# Autodesk Inventor assembly: gasienica_zlozenie
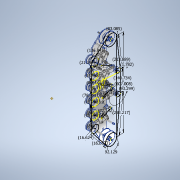
[picture p0: Inventor's stored thumbnail of the model, 180x180]
Saved by Autodesk Inventor 2020.3 (Build 243373000, 373)
## iProperties
Created: 2021-10-24
Part Number: gasienica_zlozenie
Document SubType Name: Assembly
Designer: patry
Author: patry
## Documents named in this file (31)
- C:\Users\patry\Desktop\Konar staff\Ariadna2.1\ariadna_mechanika\Obszar roboczy\Naped\Zawieszenie_v3\gasienica_zlozenie.iam
- C:\Users\patry\Desktop\Konar staff\Ariadna2.1\ariadna_mechanika\Obszar roboczy\Naped\Zawieszenie_v3\plyta_glowna_V3.ipt
- C:\Users\patry\Desktop\Konar staff\Ariadna2.1\ariadna_mechanika\Obszar roboczy\Naped\Sruby\M6_nut_5mm_MIR1.ipt
- C:\Users\patry\Desktop\Konar staff\Ariadna2.1\ariadna_mechanika\Obszar roboczy\Naped\Sruby\M6x65_MIR1.ipt
- C:\Users\patry\Desktop\Konar staff\Ariadna2.1\ariadna_mechanika\Obszar roboczy\Naped\Kola\kolo_przednie.iam
- C:\Users\patry\Desktop\Konar staff\Ariadna2.1\ariadna_mechanika\Obszar roboczy\Naped\Sruby\M5x65.ipt
- C:\Users\patry\Desktop\Konar staff\Ariadna2.1\ariadna_mechanika\Obszar roboczy\Naped\Sruby\M5_nut_5mm.ipt
- C:\Users\patry\Desktop\Konar staff\Ariadna2.1\ariadna_mechanika\Obszar roboczy\Naped\Sruby\dystans_miedzy_plytami.ipt
- C:\Users\patry\Desktop\Konar staff\Ariadna2.1\ariadna_mechanika\Obszar roboczy\Naped\Zawieszenie_v3\glowny_wahacz.ipt
- C:\Users\patry\Desktop\Konar staff\Ariadna2.1\ariadna_mechanika\Obszar roboczy\Naped\Zawieszenie_v3\ramie_1_wahacza.ipt
- C:\Users\patry\Desktop\Konar staff\Ariadna2.1\ariadna_mechanika\Obszar roboczy\Naped\Zawieszenie_v3\ramie_2_wahacza.ipt
- C:\Users\patry\Desktop\Konar staff\Ariadna2.1\ariadna_mechanika\Obszar roboczy\Naped\Zawieszenie_v3\tuleja_TUF106040.ipt
- C:\Users\patry\Desktop\Konar staff\Ariadna2.1\ariadna_mechanika\Obszar roboczy\Naped\Zawieszenie_v3\komplet_kol_V4.iam
- C:\Users\patry\Desktop\Konar staff\Ariadna2.1\ariadna_mechanika\Obszar roboczy\Naped\Sruby\M6_nut_5mm.ipt
- C:\Users\patry\Desktop\Konar staff\Ariadna2.1\ariadna_mechanika\Obszar roboczy\Naped\Sruby\M6x20.ipt
- C:\Users\patry\Desktop\Konar staff\Ariadna2.1\ariadna_mechanika\Obszar roboczy\Naped\Sruby\M6x65.ipt
- C:\Users\patry\Desktop\Konar staff\Ariadna2.1\ariadna_mechanika\Obszar roboczy\Naped\Zawieszenie_v3\independent_wheel_pair.iam
- C:\Users\patry\Desktop\Konar staff\Ariadna2.1\ariadna_mechanika\Obszar roboczy\Naped\Sruby\M6x35.ipt
- C:\Users\patry\Desktop\Konar staff\Ariadna2.1\ariadna_mechanika\Obszar roboczy\Naped\Amortyzator\Korpus.ipt
- C:\Users\patry\Desktop\Konar staff\Ariadna2.1\ariadna_mechanika\Obszar roboczy\Naped\Amortyzator\Tlok.ipt
- C:\Users\patry\Desktop\Konar staff\Ariadna2.1\ariadna_mechanika\Obszar roboczy\Naped\Amortyzator\Nakretka.ipt
- C:\Users\patry\Desktop\Konar staff\Ariadna2.1\ariadna_mechanika\Obszar roboczy\Naped\Sruby\M3_nut_5mm.ipt
- C:\Users\patry\Desktop\Konar staff\Ariadna2.1\ariadna_mechanika\Obszar roboczy\Naped\Sruby\M3x30.ipt
- C:\Users\patry\Desktop\Konar staff\Ariadna2.1\ariadna_mechanika\Obszar roboczy\Naped\Kola\single_wheel_dummie.iam
- C:\Users\patry\Desktop\Konar staff\Ariadna2.1\ariadna_mechanika\Obszar roboczy\Naped\Sruby\M5x40_threaded.ipt
- C:\Users\patry\Desktop\Konar staff\Ariadna2.1\ariadna_mechanika\Obszar roboczy\Naped\Zawieszenie_v3\glowny_wahacz_zewn.ipt
- C:\Users\patry\Desktop\Konar staff\Ariadna2.1\ariadna_mechanika\Obszar roboczy\Naped\Sruby\M8_nut_6.5mm_MIR1.ipt
- C:\Users\patry\Desktop\Konar staff\Ariadna2.1\ariadna_mechanika\Obszar roboczy\Naped\Sruby\M8x80_threaded_MIR1.ipt
- C:\Users\patry\Desktop\Konar staff\Ariadna2.1\ariadna_mechanika\Obszar roboczy\Naped\Sruby\M8_pad_MIR1.ipt
- C:\Users\patry\Desktop\Konar staff\Ariadna2.1\ariadna_mechanika\Obszar roboczy\Naped\Lozyska\608ZZ-8mm\bearings-608zz-80018-1.snapshot.1\608zz_MIR1.ipt
- C:\Users\patry\Desktop\Konar staff\Ariadna2.1\ariadna_mechanika\Obszar roboczy\Naped\Kola\kolo_napedowe.iam
## Components (177 placed, 30 different names)
1. plyta_glowna_V3:1 — Zestawiające:1, Zestawiające:2, Zestawiające:3, Zestawiające:107, Zestawiające:108, Zestawiające:110, Zestawiające:190, Zestawiające:191, Kątowe:20, Zestawiające:193, Zestawiające:260, Zestawiające:261, Zestawiające:263, Zestawiające:330, Zestawiające:331, Zestawiające:332, Zestawiające:333
2. plyta_glowna_V3:2 — Zestawiające:1, Zestawiające:2, Zestawiające:3, Zestawiające:11, Zestawiające:12, Zestawiające:19, Zestawiające:20, Zestawiające:21, Zestawiające:22, Zestawiające:26, Zestawiające:27, Zestawiające:109, Zestawiające:192, Zestawiające:262, Zestawiające:354, Równoległe:15, Kątowe:43
3. M6_nut_5mm_MIR1:1
4. M6x65_MIR1:1 — Zestawiające:11, Zestawiające:12
5. M6_nut_5mm_MIR1:2
6. M6_nut_5mm_MIR1:3
7. kolo_przednie:1 [sub-assembly]
8. M5x65:1 — Zestawiające:14, Zestawiające:15, Zestawiające:19, Zestawiające:20
9. M5_nut_5mm:1
10. dystans_miedzy_plytami:1 — Zestawiające:14, Zestawiające:15
11. M5x65:2 — Zestawiające:21, Zestawiające:22
12. M5_nut_5mm:2
13. dystans_miedzy_plytami:2
14. M5x65:3 — Zestawiające:26, Zestawiające:27
15. M5_nut_5mm:3
16. dystans_miedzy_plytami:3
17. glowny_wahacz:1
18. ramie_1_wahacza:1
19. ramie_2_wahacza:1
20. tuleja_TUF106040:1
21. tuleja_TUF106040:2
22. tuleja_TUF106040:3
23. tuleja_TUF106040:4
24. komplet_kol_V4:1 [sub-assembly] — Kątowe:43
25. glowny_wahacz:2 — Kątowe:40
26. ramie_1_wahacza:2 — Kątowe:40
27. tuleja_TUF106040:5
28. tuleja_TUF106040:6
29. ramie_2_wahacza:2
30. tuleja_TUF106040:7
31. tuleja_TUF106040:8
32. M6_nut_5mm:1
33. M6x20:1
34. M6_nut_5mm:2
35. M6_nut_5mm:3
36. M6_nut_5mm:4
37. M6x65:1 — Zestawiające:107
38. M6_nut_5mm:5
39. M6_nut_5mm:6
40. M6_nut_5mm:7
41. M6x65:2 — Zestawiające:108, Zestawiające:109
42. M6_nut_5mm:8
43. M6_nut_5mm:9
44. M6x35:1
45. M6x35:2
46. Korpus:1 — Walcowe:1
47. Tlok:1 — Walcowe:1
48. Nakretka:1
49. M3_nut_5mm:1
50. M3x30:1
51. M5_nut_5mm:4
52. M5x65:4 — Zestawiające:110
53. single_wheel_dummie:1 [sub-assembly]
54. M5_nut_5mm:5
55. M5x40_threaded:1
56. single_wheel_dummie:2 [sub-assembly]
57. M5_nut_5mm:6
58. glowny_wahacz:3
59. ramie_1_wahacza:3
60. ramie_2_wahacza:3
61. tuleja_TUF106040:9
62. tuleja_TUF106040:10
63. tuleja_TUF106040:11
64. tuleja_TUF106040:12
65. komplet_kol_V4:2 [sub-assembly] — Kątowe:20
66. glowny_wahacz:4 — Kątowe:41
67. ramie_1_wahacza:4 — Kątowe:41
68. tuleja_TUF106040:13
69. tuleja_TUF106040:14
70. ramie_2_wahacza:4
71. tuleja_TUF106040:15
72. tuleja_TUF106040:16
73. M6_nut_5mm:10
74. M6x20:2
75. M6_nut_5mm:11
76. M6_nut_5mm:12
77. M6_nut_5mm:13
78. M6x65:3 — Zestawiające:191, Zestawiające:192
79. M6_nut_5mm:14
80. M6_nut_5mm:15
81. M6_nut_5mm:16
82. M6x65:4 — Zestawiające:190
83. M6_nut_5mm:17
84. M6_nut_5mm:18
85. M6x35:3
86. M6x35:4
87. Korpus:2 — Walcowe:2
88. Tlok:2 — Walcowe:2
89. Nakretka:2
90. M3_nut_5mm:2
91. M3x30:2
92. M5_nut_5mm:7
93. M5x65:5 — Zestawiające:193
94. single_wheel_dummie:3 [sub-assembly]
95. M5_nut_5mm:8
96. M5x40_threaded:2
97. single_wheel_dummie:4 [sub-assembly]
98. M5_nut_5mm:9
99. ramie_1_wahacza:5 — Kątowe:39
100. ramie_2_wahacza:5
101. tuleja_TUF106040:17
102. tuleja_TUF106040:18
103. tuleja_TUF106040:19
104. tuleja_TUF106040:20
105. ramie_1_wahacza:6
106. tuleja_TUF106040:21
107. tuleja_TUF106040:22
108. ramie_2_wahacza:6
109. tuleja_TUF106040:23
110. tuleja_TUF106040:24
111. M6_nut_5mm:19
112. M6_nut_5mm:20
113. M6_nut_5mm:21
114. M6x65:5 — Zestawiające:260
115. M6_nut_5mm:22
116. M6_nut_5mm:23
117. M6_nut_5mm:24
118. M6x65:6 — Zestawiające:261
119. M6_nut_5mm:25 — Zestawiające:262
120. M6_nut_5mm:26
121. M6x35:5
122. M6x35:6
123. Korpus:3 — Walcowe:3
124. Tlok:3 — Walcowe:3
125. Nakretka:3
126. M3_nut_5mm:3
127. M3x30:3
128. M5_nut_5mm:10
129. M5x65:6 — Zestawiające:263
130. glowny_wahacz_zewn:1
131. glowny_wahacz_zewn:2 — Kątowe:39
132. independent_wheel_pair:1 [sub-assembly]
133. ramie_1_wahacza:7 — Kątowe:42
134. ramie_2_wahacza:7
135. tuleja_TUF106040:25
136. tuleja_TUF106040:26
137. tuleja_TUF106040:27
138. tuleja_TUF106040:28
139. ramie_1_wahacza:8
140. tuleja_TUF106040:29
141. tuleja_TUF106040:30
142. ramie_2_wahacza:8
143. tuleja_TUF106040:31
144. tuleja_TUF106040:32
145. M6_nut_5mm:27
146. M6_nut_5mm:28
147. M6_nut_5mm:29
148. M6x65:7 — Zestawiające:330
149. M6_nut_5mm:30 — Zestawiające:331
150. M6_nut_5mm:31
151. M6_nut_5mm:32
152. M6x65:8 — Zestawiające:332
153. M6_nut_5mm:33
154. M6_nut_5mm:34
155. M6x35:7
156. M6x35:8
157. Korpus:4 — Walcowe:4
158. Tlok:4 — Walcowe:4
159. Nakretka:4
160. M3_nut_5mm:4
161. M3x30:4
162. M5_nut_5mm:11
163. M5x65:7 — Zestawiające:333
164. glowny_wahacz_zewn:3
165. glowny_wahacz_zewn:4 — Kątowe:42
166. independent_wheel_pair:2 [sub-assembly]
167. M8_nut_6.5mm_MIR1:1
168. M8x80_threaded_MIR1:1
169. M8_nut_6.5mm_MIR1:2
170. M8_nut_6.5mm_MIR1:3
171. M8_pad_MIR1:1
172. M8_pad_MIR1:2
173. M8_pad_MIR1:3
174. M8_pad_MIR1:4
175. 608zz_MIR1:1
176. 608zz_MIR1:2 — Zestawiające:354, Równoległe:15
177. kolo_napedowe:1 [sub-assembly]
## Relationships (415: Mate 354, Angle 42, Flush 15, CylindricalJoint 4)
- Zestawiające:1 [Mate]: plyta_glowna_V3:1 ↔ plyta_glowna_V3:2
- Zestawiające:2 [Mate]: plyta_glowna_V3:1 ↔ plyta_glowna_V3:2
- Zestawiające:3 [Mate] (50 mm): plyta_glowna_V3:1 ↔ plyta_glowna_V3:2
- [Flush]: M6_nut_5mm_MIR1:1 ↔ M6x65_MIR1:1
- [Mate]: M6_nut_5mm_MIR1:1 ↔ M6x65_MIR1:1
- [Mate] (12 mm): M6_nut_5mm_MIR1:1 ↔ M6_nut_5mm_MIR1:2
- [Mate]: M6x65_MIR1:1 ↔ M6_nut_5mm_MIR1:2
- [Mate] (12 mm): M6x65_MIR1:1 ↔ M6_nut_5mm_MIR1:3
- [Mate]: M6x65_MIR1:1 ↔ M6_nut_5mm_MIR1:3
- [Mate]: M6x65_MIR1:1 ↔ kolo_przednie:1
- [Mate]: M6_nut_5mm_MIR1:3 ↔ kolo_przednie:1
- Zestawiające:11 [Mate]: plyta_glowna_V3:2 ↔ M6x65_MIR1:1
- Zestawiające:12 [Mate]: plyta_glowna_V3:2 ↔ M6x65_MIR1:1
- [Mate]: M5x65:1 ↔ M5_nut_5mm:1
- [Flush]: M5x65:1 ↔ M5_nut_5mm:1
- Zestawiające:14 [Mate]: M5x65:1 ↔ dystans_miedzy_plytami:1
- Zestawiające:15 [Mate] (5 mm): M5x65:1 ↔ dystans_miedzy_plytami:1
- [Mate]: M5x65:2 ↔ M5_nut_5mm:2
- [Flush]: M5x65:2 ↔ M5_nut_5mm:2
- [Mate]: M5x65:2 ↔ dystans_miedzy_plytami:2
- [Mate] (5 mm): M5x65:2 ↔ dystans_miedzy_plytami:2
- Zestawiające:19 [Mate]: plyta_glowna_V3:2 ↔ M5x65:1
- Zestawiające:20 [Mate]: plyta_glowna_V3:2 ↔ M5x65:1
- Zestawiające:21 [Mate]: plyta_glowna_V3:2 ↔ M5x65:2
- Zestawiające:22 [Mate]: plyta_glowna_V3:2 ↔ M5x65:2
- [Mate]: M5x65:3 ↔ M5_nut_5mm:3
- [Flush]: M5x65:3 ↔ M5_nut_5mm:3
- [Mate]: M5x65:3 ↔ dystans_miedzy_plytami:3
- [Mate] (5 mm): M5x65:3 ↔ dystans_miedzy_plytami:3
- Zestawiające:26 [Mate]: plyta_glowna_V3:2 ↔ M5x65:3
- Zestawiające:27 [Mate]: plyta_glowna_V3:2 ↔ M5x65:3
- [Mate]: ramie_2_wahacza:1 ↔ tuleja_TUF106040:1
- [Mate]: ramie_2_wahacza:1 ↔ tuleja_TUF106040:1
- [Mate]: ramie_2_wahacza:1 ↔ tuleja_TUF106040:2
- [Mate]: ramie_2_wahacza:1 ↔ tuleja_TUF106040:2
- [Angle] (0 deg): ramie_2_wahacza:1 ↔ tuleja_TUF106040:1
- [Angle] (0 deg): ramie_2_wahacza:1 ↔ tuleja_TUF106040:2
- [Mate]: ramie_1_wahacza:1 ↔ tuleja_TUF106040:3
- [Mate]: ramie_1_wahacza:1 ↔ tuleja_TUF106040:3
- [Angle] (0 deg): ramie_1_wahacza:1 ↔ tuleja_TUF106040:3
- [Mate]: ramie_1_wahacza:1 ↔ tuleja_TUF106040:4
- [Mate]: ramie_1_wahacza:1 ↔ tuleja_TUF106040:4
- [Angle] (0 deg): ramie_1_wahacza:1 ↔ tuleja_TUF106040:4
- [Mate]: glowny_wahacz:1 ↔ komplet_kol_V4:1
- [Mate]: komplet_kol_V4:1 ↔ glowny_wahacz:2
- [Mate]: komplet_kol_V4:1 ↔ glowny_wahacz:2
- [Mate]: glowny_wahacz:1 ↔ komplet_kol_V4:1
- [Mate]: glowny_wahacz:1 ↔ tuleja_TUF106040:4
- [Mate] (2.5 mm): glowny_wahacz:1 ↔ tuleja_TUF106040:4
- [Mate]: ramie_1_wahacza:2 ↔ tuleja_TUF106040:5
- [Mate]: ramie_1_wahacza:2 ↔ tuleja_TUF106040:5
- [Angle] (0 deg): ramie_1_wahacza:2 ↔ tuleja_TUF106040:5
- [Mate]: ramie_1_wahacza:2 ↔ tuleja_TUF106040:6
- [Mate]: ramie_1_wahacza:2 ↔ tuleja_TUF106040:6
- [Angle] (0 deg): ramie_1_wahacza:2 ↔ tuleja_TUF106040:6
- [Mate] (2.5 mm): glowny_wahacz:2 ↔ tuleja_TUF106040:6
- [Mate]: glowny_wahacz:2 ↔ tuleja_TUF106040:6
- [Mate]: tuleja_TUF106040:3 ↔ tuleja_TUF106040:5
- [Mate] (2.5 mm): glowny_wahacz:1 ↔ tuleja_TUF106040:1
- [Mate]: ramie_2_wahacza:2 ↔ tuleja_TUF106040:7
- [Mate]: ramie_2_wahacza:2 ↔ tuleja_TUF106040:7
- [Mate]: ramie_2_wahacza:2 ↔ tuleja_TUF106040:8
- [Mate]: ramie_2_wahacza:2 ↔ tuleja_TUF106040:8
- [Angle] (0 deg): ramie_2_wahacza:2 ↔ tuleja_TUF106040:7
- [Angle] (0 deg): ramie_2_wahacza:2 ↔ tuleja_TUF106040:8
- [Mate] (2.5 mm): glowny_wahacz:2 ↔ tuleja_TUF106040:7
- [Mate]: tuleja_TUF106040:2 ↔ tuleja_TUF106040:8
- [Mate]: glowny_wahacz:1 ↔ M6x20:1
- [Mate]: glowny_wahacz:2 ↔ M6x20:1
- [Mate]: M6_nut_5mm:1 ↔ M6x20:1
- [Mate]: glowny_wahacz:1 ↔ M6_nut_5mm:1
- [Mate]: ramie_1_wahacza:1 ↔ M6_nut_5mm:2
- [Mate]: ramie_2_wahacza:1 ↔ M6_nut_5mm:3
- [Mate]: M6_nut_5mm:4 ↔ M6x65:1
- [Mate] (5 mm): M6_nut_5mm:4 ↔ M6x65:1
- [Mate] (-5 mm): M6x65:1 ↔ M6_nut_5mm:5
- [Mate]: M6x65:1 ↔ M6_nut_5mm:5
- [Mate]: M6x65:1 ↔ M6_nut_5mm:6
- [Mate] (5 mm): M6_nut_5mm:5 ↔ M6_nut_5mm:6
- [Mate]: tuleja_TUF106040:3 ↔ M6x65:1
- [Mate] (9.5 mm): ramie_1_wahacza:1 ↔ M6_nut_5mm:6
- [Mate]: M6_nut_5mm:7 ↔ M6x65:2
- [Mate] (5 mm): M6_nut_5mm:7 ↔ M6x65:2
- [Mate] (-5 mm): M6x65:2 ↔ M6_nut_5mm:8
- [Mate]: M6x65:2 ↔ M6_nut_5mm:8
- [Mate]: M6x65:2 ↔ M6_nut_5mm:9
- [Mate] (5 mm): M6_nut_5mm:8 ↔ M6_nut_5mm:9
- [Mate]: tuleja_TUF106040:8 ↔ M6x65:2
- [Mate] (9.5 mm): ramie_2_wahacza:1 ↔ M6_nut_5mm:9
- [Mate]: tuleja_TUF106040:1 ↔ M6x35:1
- [Mate]: ramie_2_wahacza:2 ↔ M6x35:1
- [Mate]: M6_nut_5mm:3 ↔ M6x35:1
- [Mate]: glowny_wahacz:1 ↔ M6x35:2
- [Mate]: ramie_1_wahacza:2 ↔ M6x35:2
- [Mate]: M6_nut_5mm:2 ↔ M6x35:2
- [Mate]: Korpus:1 ↔ Tlok:1
- [Angle] (0 deg): Korpus:1 ↔ Tlok:1
- [Mate]: Korpus:1 ↔ Nakretka:1
- [Mate] (5 mm): Korpus:1 ↔ Nakretka:1
- Walcowe:1 [CylindricalJoint]: Korpus:1 ↔ Tlok:1
- [Mate]: ramie_1_wahacza:2 ↔ Tlok:1
- [Mate] (7.5 mm): ramie_1_wahacza:2 ↔ Tlok:1
- [Mate]: ramie_1_wahacza:2 ↔ M3x30:1
- [Mate]: ramie_1_wahacza:2 ↔ M3x30:1
- [Mate]: M3_nut_5mm:1 ↔ M3x30:1
- [Mate]: ramie_1_wahacza:1 ↔ M3_nut_5mm:1
- [Mate]: Korpus:1 ↔ M5x65:4
- [Mate]: M5_nut_5mm:4 ↔ M5x65:4
- [Flush]: M6x65:2 ↔ M5x65:4
- [Flush]: M6_nut_5mm:8 ↔ M5_nut_5mm:4
- [Mate]: tuleja_TUF106040:7 ↔ M6x35:1
- [Mate]: glowny_wahacz:1 ↔ M6x35:1
- [Mate]: glowny_wahacz:1 ↔ glowny_wahacz:2
- [Mate]: glowny_wahacz:1 ↔ M5x40_threaded:1
- [Flush] (13.5 mm): glowny_wahacz:1 ↔ M5x40_threaded:1
- [Mate]: single_wheel_dummie:1 ↔ M5x40_threaded:1
- [Mate] (1 mm): glowny_wahacz:1 ↔ single_wheel_dummie:1
- [Mate]: M5x40_threaded:1 ↔ single_wheel_dummie:2
- [Mate] (1 mm): glowny_wahacz:2 ↔ single_wheel_dummie:2
- [Mate]: M5_nut_5mm:5 ↔ M5x40_threaded:1
- [Mate]: single_wheel_dummie:1 ↔ M5_nut_5mm:5
- [Mate]: M5x40_threaded:1 ↔ M5_nut_5mm:6
- [Mate]: single_wheel_dummie:2 ↔ M5_nut_5mm:6
- Zestawiające:107 [Mate]: plyta_glowna_V3:1 ↔ M6x65:1
- Zestawiające:108 [Mate]: plyta_glowna_V3:1 ↔ M6x65:2
- Zestawiające:109 [Mate]: plyta_glowna_V3:2 ↔ M6x65:2
- Zestawiające:110 [Mate]: plyta_glowna_V3:1 ↔ M5x65:4
- [Mate]: ramie_2_wahacza:3 ↔ tuleja_TUF106040:9
- [Mate]: ramie_2_wahacza:3 ↔ tuleja_TUF106040:9
- [Mate]: ramie_2_wahacza:3 ↔ tuleja_TUF106040:10
- [Mate]: ramie_2_wahacza:3 ↔ tuleja_TUF106040:10
- [Angle] (0 deg): ramie_2_wahacza:3 ↔ tuleja_TUF106040:9
- [Angle] (0 deg): ramie_2_wahacza:3 ↔ tuleja_TUF106040:10
- [Mate]: ramie_1_wahacza:3 ↔ tuleja_TUF106040:11
- [Mate]: ramie_1_wahacza:3 ↔ tuleja_TUF106040:11
- [Angle] (0 deg): ramie_1_wahacza:3 ↔ tuleja_TUF106040:11
- [Mate]: ramie_1_wahacza:3 ↔ tuleja_TUF106040:12
- [Mate]: ramie_1_wahacza:3 ↔ tuleja_TUF106040:12
- [Angle] (0 deg): ramie_1_wahacza:3 ↔ tuleja_TUF106040:12
- [Mate]: glowny_wahacz:3 ↔ komplet_kol_V4:2
- [Mate]: komplet_kol_V4:2 ↔ glowny_wahacz:4
- [Mate]: komplet_kol_V4:2 ↔ glowny_wahacz:4
- [Mate]: glowny_wahacz:3 ↔ komplet_kol_V4:2
- [Mate]: glowny_wahacz:3 ↔ tuleja_TUF106040:12
- [Mate] (2.5 mm): glowny_wahacz:3 ↔ tuleja_TUF106040:12
- [Mate]: ramie_1_wahacza:4 ↔ tuleja_TUF106040:13
- [Mate]: ramie_1_wahacza:4 ↔ tuleja_TUF106040:13
- [Angle] (0 deg): ramie_1_wahacza:4 ↔ tuleja_TUF106040:13
- [Mate]: ramie_1_wahacza:4 ↔ tuleja_TUF106040:14
- [Mate]: ramie_1_wahacza:4 ↔ tuleja_TUF106040:14
- [Angle] (0 deg): ramie_1_wahacza:4 ↔ tuleja_TUF106040:14
- [Mate] (2.5 mm): glowny_wahacz:4 ↔ tuleja_TUF106040:14
- [Mate]: glowny_wahacz:4 ↔ tuleja_TUF106040:14
- [Mate]: tuleja_TUF106040:11 ↔ tuleja_TUF106040:13
- [Mate] (2.5 mm): glowny_wahacz:3 ↔ tuleja_TUF106040:9
- [Mate]: ramie_2_wahacza:4 ↔ tuleja_TUF106040:15
- [Mate]: ramie_2_wahacza:4 ↔ tuleja_TUF106040:15
- [Mate]: ramie_2_wahacza:4 ↔ tuleja_TUF106040:16
- [Mate]: ramie_2_wahacza:4 ↔ tuleja_TUF106040:16
- [Angle] (0 deg): ramie_2_wahacza:4 ↔ tuleja_TUF106040:15
- [Angle] (0 deg): ramie_2_wahacza:4 ↔ tuleja_TUF106040:16
- [Mate] (2.5 mm): glowny_wahacz:4 ↔ tuleja_TUF106040:15
- [Mate]: tuleja_TUF106040:10 ↔ tuleja_TUF106040:16
- [Mate]: glowny_wahacz:3 ↔ M6x20:2
- [Mate]: glowny_wahacz:4 ↔ M6x20:2
- [Mate]: M6_nut_5mm:10 ↔ M6x20:2
- [Mate]: glowny_wahacz:3 ↔ M6_nut_5mm:10
- [Mate]: ramie_1_wahacza:3 ↔ M6_nut_5mm:11
- [Mate]: ramie_2_wahacza:3 ↔ M6_nut_5mm:12
- [Mate]: M6_nut_5mm:13 ↔ M6x65:3
- [Mate] (5 mm): M6_nut_5mm:13 ↔ M6x65:3
- [Mate] (-5 mm): M6x65:3 ↔ M6_nut_5mm:14
- [Mate]: M6x65:3 ↔ M6_nut_5mm:14
- [Mate]: M6x65:3 ↔ M6_nut_5mm:15
- [Mate] (5 mm): M6_nut_5mm:14 ↔ M6_nut_5mm:15
- [Mate]: tuleja_TUF106040:11 ↔ M6x65:3
- [Mate] (9.5 mm): ramie_1_wahacza:3 ↔ M6_nut_5mm:15
- [Mate]: M6_nut_5mm:16 ↔ M6x65:4
- [Mate] (5 mm): M6_nut_5mm:16 ↔ M6x65:4
- [Mate] (-5 mm): M6x65:4 ↔ M6_nut_5mm:17
- [Mate]: M6x65:4 ↔ M6_nut_5mm:17
- [Mate]: M6x65:4 ↔ M6_nut_5mm:18
- [Mate] (5 mm): M6_nut_5mm:17 ↔ M6_nut_5mm:18
- [Mate]: tuleja_TUF106040:16 ↔ M6x65:4
- [Mate] (9.5 mm): ramie_2_wahacza:3 ↔ M6_nut_5mm:18
- [Mate]: tuleja_TUF106040:9 ↔ M6x35:3
- [Mate]: ramie_2_wahacza:4 ↔ M6x35:3
- [Mate]: M6_nut_5mm:12 ↔ M6x35:3
- [Mate]: glowny_wahacz:3 ↔ M6x35:4
- [Mate]: ramie_1_wahacza:4 ↔ M6x35:4
- [Mate]: M6_nut_5mm:11 ↔ M6x35:4
- [Mate]: Korpus:2 ↔ Tlok:2
- [Angle] (0 deg): Korpus:2 ↔ Tlok:2
- [Mate]: Korpus:2 ↔ Nakretka:2
- [Mate] (5 mm): Korpus:2 ↔ Nakretka:2
- Walcowe:2 [CylindricalJoint]: Korpus:2 ↔ Tlok:2
- [Mate]: ramie_1_wahacza:4 ↔ Tlok:2
- [Mate] (7.5 mm): ramie_1_wahacza:4 ↔ Tlok:2
- [Mate]: ramie_1_wahacza:4 ↔ M3x30:2
- [Mate]: ramie_1_wahacza:4 ↔ M3x30:2
- [Mate]: M3_nut_5mm:2 ↔ M3x30:2
- [Mate]: ramie_1_wahacza:3 ↔ M3_nut_5mm:2
- [Mate]: Korpus:2 ↔ M5x65:5
- [Mate]: M5_nut_5mm:7 ↔ M5x65:5
- [Flush]: M6x65:4 ↔ M5x65:5
- [Flush]: M6_nut_5mm:17 ↔ M5_nut_5mm:7
- [Mate]: tuleja_TUF106040:15 ↔ M6x35:3
- [Mate]: glowny_wahacz:3 ↔ M6x35:3
- [Mate]: glowny_wahacz:3 ↔ glowny_wahacz:4
- [Mate]: glowny_wahacz:3 ↔ M5x40_threaded:2
- [Flush] (13.5 mm): glowny_wahacz:3 ↔ M5x40_threaded:2
- [Mate]: single_wheel_dummie:3 ↔ M5x40_threaded:2
- [Mate] (1 mm): glowny_wahacz:3 ↔ single_wheel_dummie:3
- [Mate]: M5x40_threaded:2 ↔ single_wheel_dummie:4
- [Mate] (1 mm): glowny_wahacz:4 ↔ single_wheel_dummie:4
- [Mate]: M5_nut_5mm:8 ↔ M5x40_threaded:2
- [Mate]: single_wheel_dummie:3 ↔ M5_nut_5mm:8
- [Mate]: M5x40_threaded:2 ↔ M5_nut_5mm:9
- [Mate]: single_wheel_dummie:4 ↔ M5_nut_5mm:9
- Zestawiające:190 [Mate]: plyta_glowna_V3:1 ↔ M6x65:4
- Zestawiające:191 [Mate]: plyta_glowna_V3:1 ↔ M6x65:3
- Zestawiające:192 [Mate]: plyta_glowna_V3:2 ↔ M6x65:3
- Kątowe:20 [Angle] (0 deg): plyta_glowna_V3:1 ↔ komplet_kol_V4:2
- Zestawiające:193 [Mate]: plyta_glowna_V3:1 ↔ M5x65:5
- [Mate]: ramie_2_wahacza:5 ↔ tuleja_TUF106040:17
- [Mate]: ramie_2_wahacza:5 ↔ tuleja_TUF106040:17
- [Mate]: ramie_2_wahacza:5 ↔ tuleja_TUF106040:18
- [Mate]: ramie_2_wahacza:5 ↔ tuleja_TUF106040:18
- [Angle] (0 deg): ramie_2_wahacza:5 ↔ tuleja_TUF106040:17
- [Angle] (0 deg): ramie_2_wahacza:5 ↔ tuleja_TUF106040:18
- [Mate]: ramie_1_wahacza:5 ↔ tuleja_TUF106040:19
- [Mate]: ramie_1_wahacza:5 ↔ tuleja_TUF106040:19
- [Angle] (0 deg): ramie_1_wahacza:5 ↔ tuleja_TUF106040:19
- [Mate]: ramie_1_wahacza:5 ↔ tuleja_TUF106040:20
- [Mate]: ramie_1_wahacza:5 ↔ tuleja_TUF106040:20
- [Angle] (0 deg): ramie_1_wahacza:5 ↔ tuleja_TUF106040:20
- [Mate]: ramie_1_wahacza:6 ↔ tuleja_TUF106040:21
- [Mate]: ramie_1_wahacza:6 ↔ tuleja_TUF106040:21
- [Angle] (0 deg): ramie_1_wahacza:6 ↔ tuleja_TUF106040:21
- [Mate]: ramie_1_wahacza:6 ↔ tuleja_TUF106040:22
- [Mate]: ramie_1_wahacza:6 ↔ tuleja_TUF106040:22
- [Angle] (0 deg): ramie_1_wahacza:6 ↔ tuleja_TUF106040:22
- [Mate]: tuleja_TUF106040:19 ↔ tuleja_TUF106040:21
- [Mate]: ramie_2_wahacza:6 ↔ tuleja_TUF106040:23
- [Mate]: ramie_2_wahacza:6 ↔ tuleja_TUF106040:23
- [Mate]: ramie_2_wahacza:6 ↔ tuleja_TUF106040:24
- [Mate]: ramie_2_wahacza:6 ↔ tuleja_TUF106040:24
- [Angle] (0 deg): ramie_2_wahacza:6 ↔ tuleja_TUF106040:23
- [Angle] (0 deg): ramie_2_wahacza:6 ↔ tuleja_TUF106040:24
- [Mate]: tuleja_TUF106040:18 ↔ tuleja_TUF106040:24
- [Mate]: ramie_1_wahacza:5 ↔ M6_nut_5mm:19
- [Mate]: ramie_2_wahacza:5 ↔ M6_nut_5mm:20
- [Mate]: M6_nut_5mm:21 ↔ M6x65:5
- [Mate] (5 mm): M6_nut_5mm:21 ↔ M6x65:5
- [Mate] (-5 mm): M6x65:5 ↔ M6_nut_5mm:22
- [Mate]: M6x65:5 ↔ M6_nut_5mm:22
- [Mate]: M6x65:5 ↔ M6_nut_5mm:23
- [Mate] (5 mm): M6_nut_5mm:22 ↔ M6_nut_5mm:23
- [Mate]: tuleja_TUF106040:19 ↔ M6x65:5
- [Mate] (4.5 mm): ramie_1_wahacza:5 ↔ M6_nut_5mm:23
- [Mate]: M6_nut_5mm:24 ↔ M6x65:6
- [Mate] (5 mm): M6_nut_5mm:24 ↔ M6x65:6
- [Mate] (-5 mm): M6x65:6 ↔ M6_nut_5mm:25
- [Mate]: M6x65:6 ↔ M6_nut_5mm:25
- [Mate]: M6x65:6 ↔ M6_nut_5mm:26
- [Mate] (5 mm): M6_nut_5mm:25 ↔ M6_nut_5mm:26
- [Mate]: tuleja_TUF106040:24 ↔ M6x65:6
- [Mate] (4.5 mm): ramie_2_wahacza:5 ↔ M6_nut_5mm:26
- [Mate]: tuleja_TUF106040:17 ↔ M6x35:5
- [Mate]: ramie_2_wahacza:6 ↔ M6x35:5
- [Mate]: M6_nut_5mm:20 ↔ M6x35:5
- [Mate]: ramie_1_wahacza:6 ↔ M6x35:6
- [Mate]: M6_nut_5mm:19 ↔ M6x35:6
- [Mate]: Korpus:3 ↔ Tlok:3
- [Angle] (0 deg): Korpus:3 ↔ Tlok:3
- [Mate]: Korpus:3 ↔ Nakretka:3
- [Mate] (5 mm): Korpus:3 ↔ Nakretka:3
- Walcowe:3 [CylindricalJoint]: Korpus:3 ↔ Tlok:3
- [Mate]: ramie_1_wahacza:6 ↔ Tlok:3
- [Mate] (7.5 mm): ramie_1_wahacza:6 ↔ Tlok:3
- [Mate]: ramie_1_wahacza:6 ↔ M3x30:3
- [Mate]: ramie_1_wahacza:6 ↔ M3x30:3
- [Mate]: M3_nut_5mm:3 ↔ M3x30:3
- [Mate]: ramie_1_wahacza:5 ↔ M3_nut_5mm:3
- [Mate]: Korpus:3 ↔ M5x65:6
- [Mate]: M5_nut_5mm:10 ↔ M5x65:6
- [Flush]: M6x65:6 ↔ M5x65:6
- [Flush]: M6_nut_5mm:25 ↔ M5_nut_5mm:10
- [Mate]: tuleja_TUF106040:23 ↔ M6x35:5
- [Mate]: M6x35:5 ↔ glowny_wahacz_zewn:1
- [Mate]: M6x35:5 ↔ glowny_wahacz_zewn:2
- [Mate] (2.5 mm): tuleja_TUF106040:17 ↔ glowny_wahacz_zewn:2
- [Mate] (2.5 mm): tuleja_TUF106040:23 ↔ glowny_wahacz_zewn:1
- [Mate]: glowny_wahacz_zewn:1 ↔ glowny_wahacz_zewn:2
- [Mate]: M6x35:6 ↔ glowny_wahacz_zewn:2
- [Mate]: tuleja_TUF106040:20 ↔ M6x35:6
- [Mate]: tuleja_TUF106040:22 ↔ M6x35:6
- [Mate] (2.5 mm): tuleja_TUF106040:20 ↔ glowny_wahacz_zewn:2
- [Mate] (2.5 mm): tuleja_TUF106040:22 ↔ glowny_wahacz_zewn:1
- [Mate] (7 mm): glowny_wahacz_zewn:1 ↔ glowny_wahacz_zewn:2
- [Mate]: glowny_wahacz_zewn:1 ↔ independent_wheel_pair:1
- [Mate]: glowny_wahacz_zewn:1 ↔ independent_wheel_pair:1
- Zestawiające:260 [Mate]: plyta_glowna_V3:1 ↔ M6x65:5
- Zestawiające:261 [Mate]: plyta_glowna_V3:1 ↔ M6x65:6
- Zestawiające:262 [Mate]: plyta_glowna_V3:2 ↔ M6_nut_5mm:25
- Zestawiające:263 [Mate]: plyta_glowna_V3:1 ↔ M5x65:6
- [Mate]: ramie_2_wahacza:7 ↔ tuleja_TUF106040:25
- [Mate]: ramie_2_wahacza:7 ↔ tuleja_TUF106040:25
- [Mate]: ramie_2_wahacza:7 ↔ tuleja_TUF106040:26
- [Mate]: ramie_2_wahacza:7 ↔ tuleja_TUF106040:26
- [Angle] (0 deg): ramie_2_wahacza:7 ↔ tuleja_TUF106040:25
- [Angle] (0 deg): ramie_2_wahacza:7 ↔ tuleja_TUF106040:26
- [Mate]: ramie_1_wahacza:7 ↔ tuleja_TUF106040:27
- [Mate]: ramie_1_wahacza:7 ↔ tuleja_TUF106040:27
- [Angle] (0 deg): ramie_1_wahacza:7 ↔ tuleja_TUF106040:27
- [Mate]: ramie_1_wahacza:7 ↔ tuleja_TUF106040:28
- [Mate]: ramie_1_wahacza:7 ↔ tuleja_TUF106040:28
- [Angle] (0 deg): ramie_1_wahacza:7 ↔ tuleja_TUF106040:28
- [Mate]: ramie_1_wahacza:8 ↔ tuleja_TUF106040:29
- [Mate]: ramie_1_wahacza:8 ↔ tuleja_TUF106040:29
- [Angle] (0 deg): ramie_1_wahacza:8 ↔ tuleja_TUF106040:29
- [Mate]: ramie_1_wahacza:8 ↔ tuleja_TUF106040:30
- [Mate]: ramie_1_wahacza:8 ↔ tuleja_TUF106040:30
- [Angle] (0 deg): ramie_1_wahacza:8 ↔ tuleja_TUF106040:30
- [Mate]: tuleja_TUF106040:27 ↔ tuleja_TUF106040:29
- [Mate]: ramie_2_wahacza:8 ↔ tuleja_TUF106040:31
- [Mate]: ramie_2_wahacza:8 ↔ tuleja_TUF106040:31
- [Mate]: ramie_2_wahacza:8 ↔ tuleja_TUF106040:32
- [Mate]: ramie_2_wahacza:8 ↔ tuleja_TUF106040:32
- [Angle] (0 deg): ramie_2_wahacza:8 ↔ tuleja_TUF106040:31
- [Angle] (0 deg): ramie_2_wahacza:8 ↔ tuleja_TUF106040:32
- [Mate]: tuleja_TUF106040:26 ↔ tuleja_TUF106040:32
- [Mate]: ramie_1_wahacza:7 ↔ M6_nut_5mm:27
- [Mate]: ramie_2_wahacza:7 ↔ M6_nut_5mm:28
- [Mate]: M6_nut_5mm:29 ↔ M6x65:7
- [Mate] (5 mm): M6_nut_5mm:29 ↔ M6x65:7
- [Mate] (-5 mm): M6x65:7 ↔ M6_nut_5mm:30
- [Mate]: M6x65:7 ↔ M6_nut_5mm:30
- [Mate]: M6x65:7 ↔ M6_nut_5mm:31
- [Mate] (5 mm): M6_nut_5mm:30 ↔ M6_nut_5mm:31
- [Mate]: tuleja_TUF106040:27 ↔ M6x65:7
- [Mate] (9.5 mm): ramie_1_wahacza:7 ↔ M6_nut_5mm:31
- [Mate]: M6_nut_5mm:32 ↔ M6x65:8
- [Mate] (5 mm): M6_nut_5mm:32 ↔ M6x65:8
- [Mate] (-5 mm): M6x65:8 ↔ M6_nut_5mm:33
- [Mate]: M6x65:8 ↔ M6_nut_5mm:33
- [Mate]: M6x65:8 ↔ M6_nut_5mm:34
- [Mate] (5 mm): M6_nut_5mm:33 ↔ M6_nut_5mm:34
- [Mate]: tuleja_TUF106040:32 ↔ M6x65:8
- [Mate] (9.5 mm): ramie_2_wahacza:7 ↔ M6_nut_5mm:34
- [Mate]: tuleja_TUF106040:25 ↔ M6x35:7
- [Mate]: ramie_2_wahacza:8 ↔ M6x35:7
- [Mate]: M6_nut_5mm:28 ↔ M6x35:7
- [Mate]: ramie_1_wahacza:8 ↔ M6x35:8
- [Mate]: M6_nut_5mm:27 ↔ M6x35:8
- [Mate]: Korpus:4 ↔ Tlok:4
- [Angle] (0 deg): Korpus:4 ↔ Tlok:4
- [Mate]: Korpus:4 ↔ Nakretka:4
- [Mate] (5 mm): Korpus:4 ↔ Nakretka:4
- Walcowe:4 [CylindricalJoint]: Korpus:4 ↔ Tlok:4
- [Mate]: ramie_1_wahacza:8 ↔ Tlok:4
- [Mate] (7.5 mm): ramie_1_wahacza:8 ↔ Tlok:4
- [Mate]: ramie_1_wahacza:8 ↔ M3x30:4
- [Mate]: ramie_1_wahacza:8 ↔ M3x30:4
- [Mate]: M3_nut_5mm:4 ↔ M3x30:4
- [Mate]: ramie_1_wahacza:7 ↔ M3_nut_5mm:4
- [Mate]: Korpus:4 ↔ M5x65:7
- [Mate]: M5_nut_5mm:11 ↔ M5x65:7
- [Flush]: M6x65:8 ↔ M5x65:7
- [Flush]: M6_nut_5mm:33 ↔ M5_nut_5mm:11
- [Mate]: tuleja_TUF106040:31 ↔ M6x35:7
- [Mate]: M6x35:7 ↔ glowny_wahacz_zewn:3
- [Mate]: M6x35:7 ↔ glowny_wahacz_zewn:4
- [Mate] (2.5 mm): tuleja_TUF106040:25 ↔ glowny_wahacz_zewn:4
- [Mate] (2.5 mm): tuleja_TUF106040:31 ↔ glowny_wahacz_zewn:3
- [Mate]: glowny_wahacz_zewn:3 ↔ glowny_wahacz_zewn:4
- [Mate]: M6x35:8 ↔ glowny_wahacz_zewn:4
- [Mate]: tuleja_TUF106040:28 ↔ M6x35:8
- [Mate]: tuleja_TUF106040:30 ↔ M6x35:8
- [Mate] (2.5 mm): tuleja_TUF106040:28 ↔ glowny_wahacz_zewn:4
- [Mate] (2.5 mm): tuleja_TUF106040:30 ↔ glowny_wahacz_zewn:3
- [Mate] (7 mm): glowny_wahacz_zewn:3 ↔ glowny_wahacz_zewn:4
- [Mate]: glowny_wahacz_zewn:3 ↔ independent_wheel_pair:2
- [Mate]: glowny_wahacz_zewn:3 ↔ independent_wheel_pair:2
- Zestawiające:330 [Mate]: plyta_glowna_V3:1 ↔ M6x65:7
- Zestawiające:331 [Mate]: plyta_glowna_V3:1 ↔ M6_nut_5mm:30
- Zestawiające:332 [Mate]: plyta_glowna_V3:1 ↔ M6x65:8
- Zestawiające:333 [Mate]: plyta_glowna_V3:1 ↔ M5x65:7
- [Mate]: M8_nut_6.5mm_MIR1:1 ↔ M8x80_threaded_MIR1:1
- [Mate]: M8x80_threaded_MIR1:1 ↔ M8_nut_6.5mm_MIR1:2
- [Mate]: M8x80_threaded_MIR1:1 ↔ M8_nut_6.5mm_MIR1:3
- [Mate]: M8_nut_6.5mm_MIR1:1 ↔ M8_pad_MIR1:1
- [Mate] (7 mm): M8x80_threaded_MIR1:1 ↔ M8_pad_MIR1:1
- [Mate]: M8x80_threaded_MIR1:1 ↔ M8_pad_MIR1:1
- [Mate]: M8_nut_6.5mm_MIR1:1 ↔ M8_pad_MIR1:2
- [Mate]: M8x80_threaded_MIR1:1 ↔ M8_pad_MIR1:2
- [Mate] (7 mm): M8_nut_6.5mm_MIR1:2 ↔ M8_pad_MIR1:3
- [Mate]: M8_nut_6.5mm_MIR1:3 ↔ M8_pad_MIR1:3
- [Mate]: M8x80_threaded_MIR1:1 ↔ M8_pad_MIR1:3
- [Mate]: M8_nut_6.5mm_MIR1:3 ↔ M8_pad_MIR1:4
- [Mate] (31 mm): M8_pad_MIR1:2 ↔ M8_pad_MIR1:4
- [Mate]: M8x80_threaded_MIR1:1 ↔ M8_pad_MIR1:4
- [Mate]: M8x80_threaded_MIR1:1 ↔ 608zz_MIR1:1
- [Mate]: M8_nut_6.5mm_MIR1:2 ↔ 608zz_MIR1:1
- [Mate]: M8x80_threaded_MIR1:1 ↔ 608zz_MIR1:2
- [Mate]: M8x80_threaded_MIR1:1 ↔ 608zz_MIR1:2
- [Mate]: M8x80_threaded_MIR1:1 ↔ kolo_napedowe:1
- [Mate]: M8_pad_MIR1:2 ↔ kolo_napedowe:1
- Zestawiające:354 [Mate]: plyta_glowna_V3:2 ↔ 608zz_MIR1:2
- Równoległe:15 [Flush] (1 mm): plyta_glowna_V3:2 ↔ 608zz_MIR1:2
- Kątowe:39 [Angle] (108 deg): ramie_1_wahacza:5 ↔ glowny_wahacz_zewn:2
- Kątowe:40 [Angle] (108 deg): glowny_wahacz:2 ↔ ramie_1_wahacza:2
- Kątowe:41 [Angle] (108 deg): glowny_wahacz:4 ↔ ramie_1_wahacza:4
- Kątowe:42 [Angle] (108 deg): ramie_1_wahacza:7 ↔ glowny_wahacz_zewn:4
- Kątowe:43 [Angle] (0 deg): plyta_glowna_V3:2 ↔ komplet_kol_V4:1
## Named parameters: d47_d24 = 0 mm, d48_d25 = 0 mm, d17_d47_d24 = 0 mm, d18_d48_d25 = 0 mm, d19_d15 = 0 mm, d20_d16 = 5 mm, d25_d17_d47_d24 = 0 mm, d26_d18_d48_d25 = 0 mm, d27_d19_d15 = 0 mm, d28_d20_d16 = 5 mm, d329_d0 = 0 mm, d330_d1 = 0 mm, d331_d2 = 0 mm, d86_d0 = 0 mm, d87_d1 = 0 deg, d88_d3 = 0 mm, d89_d4 = 5 mm, d90_d5 = 0 deg, d69_d66 = 5 mm, d70_d61 = 0 mm, d71_d62 = 5 mm, d72_d63 = -5 mm, d73_d64 = 0 mm, d74_d65 = 0 mm, d383_d77 = 0 mm, d384_d78 = 0 mm, d385_d79 = 0 mm, d386_d80 = 0 mm, d388_d82 = 0 mm, d83_d6 = 0 mm, d84_d7 = -12.85796 mm, d85_d8 = -15 mm, d398_d11 = 0 deg, d399_d22 = 0 mm, d400_d23 = 0 mm, d401_d24 = 0 mm, d29_d6 = 0 mm, d30_d7 = 0 mm, d31_d8 = 0 deg, d32_d9 = 0 mm, d33_d10 = 0 mm, d34_d11 = 0 deg, d40_d3 = 0 mm, d41_d4 = 0 deg, d42_d5 = 0 deg, d43_d0 = 0 mm, d44_d1 = 0 mm, d45_d2 = 0 mm, d429_d0 = 0 mm, d430_d1 = 0 mm, d431_d2 = 0 mm, d432_d3 = 0 mm, d433_d4 = 0 deg, d434_d105 = 13.5 mm, d435_d106 = 0 mm, d436_d107 = 1 mm, d437_d108 = 0 mm, d438_d109 = 1 mm, d439_d110 = 0 mm, d440_d111 = 0 mm, d441_d112 = 0 mm, d442_d113 = 0 mm, d443_d86_d0 = 0 mm, d444_d87_d1 = 0 deg, d445_d88_d3 = 0 mm, d446_d89_d4 = 5 mm, d447_d90_d5 = 0 deg, d448_d91 = 0 mm, d449_d92 = 7.5 mm, d450_d93 = 0 mm, d451_d94 = 0 mm, d452_d95 = 0 mm, d453_d96 = 0 mm, d454_d97 = 0 mm, d455_d98 = 0 mm, d456_d99 = 0 mm, d457_d100 = 0 mm, d458_d101 = 0 mm, d459_d102 = 0 mm, d460_d103 = 0 mm, d461_d104 = 0 mm, d462_d50 = 0 mm, d463_d51 = 0 mm, d464_d52 = 0 mm, d465_d56 = 0 mm, d466_d60 = 0 mm, d467_d61 = 0 mm, d468_d62 = 5 mm, d469_d63 = -5 mm, d470_d64 = 0 mm, d471_d65 = 0 mm, d472_d66 = 5 mm, d473_d67 = 0 mm, d474_d68 = 9.5 mm, d475_d69_d66 = 5 mm, d476_d70_d61 = 0 mm, d477_d71_d62 = 5 mm, d478_d72_d63 = -5 mm, d479_d73_d64 = 0 mm, d480_d74_d65 = 0 mm, d481_d75 = 0 mm, d482_d76 = 9.5 mm, d483_d77 = 0 mm, d484_d78 = 0 mm, d485_d79 = 0 mm, d486_d80 = 0 mm, d487_d81 = 0 mm, d488_d82 = 0 mm, d489_d83_d6 = 0 mm, d490_d84_d7 = -12.85796 mm, d491_d85_d8 = -15 mm, d492_d5 = 0 deg, d493_d6 = 0 mm, d494_d7 = 0 mm, d495_d8 = 0 deg, d496_d9 = 0 mm, d497_d10 = 0 mm, d498_d11 = 0 deg, d499_d22 = 0 mm, d500_d23 = 0 mm, d501_d24 = 0 mm, d502_d25 = 0 mm, d503_d27 = 0 mm, d504_d28 = 2.5 mm, d505_d29_d6 = 0 mm, d506_d30_d7 = 0 mm, d507_d31_d8 = 0 deg, d508_d32_d9 = 0 mm, d509_d33_d10 = 0 mm, d510_d34_d11 = 0 deg, d511_d35 = 2.5 mm, d512_d36 = 0 mm, d513_d37 = 0 mm, d514_d38 = 2.5 mm, d515_d40_d3 = 0 mm, d516_d41_d4 = 0 deg, d517_d42_d5 = 0 deg, d518_d43_d0 = 0 mm, d519_d44_d1 = 0 mm, d520_d45_d2 = 0 mm, d521_d46 = 2.5 mm, d522_d48 = 0 mm, d523_d49 = 0 mm, d541_d91 = 0 mm, d542_d92 = 7.5 mm, d543_d93 = 0 mm, d544_d94 = 0 mm, d545_d95 = 0 mm, d546_d96 = 0 mm, d547_d97 = 0 mm, d548_d98 = 0 mm, d549_d99 = 0 mm, d550_d100 = 0 mm, d551_d101 = 0 mm, d553_d56 = 0 mm, d554_d60 = 0 mm, d555_d61 = 0 mm, d556_d62 = 5 mm, d557_d63 = -5 mm, d558_d64 = 0 mm, d559_d65 = 0 mm, d560_d66 = 5 mm, d561_d67 = 0 mm, d562_d68 = 4.5 mm, d563_d69_d66 = 5 mm, d564_d70_d61 = 0 mm, d565_d71_d62 = 5 mm, d566_d72_d63 = -5 mm, d567_d73_d64 = 0 mm, d568_d74_d65 = 0 mm, d569_d75 = 0 mm, d570_d76 = 4.5 mm, d571_d77 = 0 mm, d572_d78 = 0 mm, d573_d79 = 0 mm, d574_d81 = 0 mm, d575_d82 = 0 mm, d576_d83_d6 = 0 mm, d577_d84_d7 = -12.858 mm, d578_d85_d8 = -15 mm, d579_d86_d0 = 0 mm, d580_d87_d1 = 0 deg, d581_d88_d3 = 0 mm, d582_d89_d4 = 5 mm, d583_d90_d5 = 0 deg, d584_d5 = 0 deg, d585_d6 = 0 mm, d586_d7 = 0 mm, d587_d8 = 0 deg, d588_d9 = 0 mm, d589_d10 = 0 mm, d590_d11 = 0 deg, d591_d29_d6 = 0 mm, d592_d30_d7 = 0 mm, d593_d31_d8 = 0 deg, d594_d32_d9 = 0 mm, d595_d33_d10 = 0 mm, d596_d34_d11 = 0 deg, d597_d37 = 0 mm, d598_d40_d3 = 0 mm, d599_d41_d4 = 0 deg, d600_d42_d5 = 0 deg, d601_d43_d0 = 0 mm, d602_d44_d1 = 0 mm, d603_d45_d2 = 0 mm, d604_d48 = 0 mm, d605_d0 = 0 mm, d606_d1 = 0 mm, d607_d2 = 0 mm, d608_d3 = 0 mm, d609_d4 = 0 deg, d614_d115 = 0 mm, d615_d116 = 2.5 mm, d616_d117 = 2.5 mm, d617_d118 = 0 mm, d618_d119 = 0 mm, d619_d120 = 0 mm, d620_d121 = 0 mm, d621_d122 = 2.5 mm, d622_d123 = 2.5 mm, d623_d124 = 7 mm, d624_d125 = 0 mm, d625_d126 = 0 mm, d626_d91 = 0 mm, d627_d92 = 7.5 mm, d628_d93 = 0 mm, d629_d94 = 0 mm, d630_d95 = 0 mm, d631_d96 = 0 mm, d632_d97 = 0 mm, d633_d98 = 0 mm, d634_d99 = 0 mm, d635_d100 = 0 mm, d636_d101 = 0 mm, d637_d114 = 0 mm, d638_d56 = 0 mm, d639_d60 = 0 mm, d640_d61 = 0 mm, d641_d62 = 5 mm, d642_d63 = -5 mm, d643_d64 = 0 mm, d644_d65 = 0 mm, d645_d66 = 5 mm, d646_d67 = 0 mm, d647_d68 = 9.5 mm, d648_d69_d66 = 5 mm, d649_d70_d61 = 0 mm, d650_d71_d62 = 5 mm, d651_d72_d63 = -5 mm, d652_d73_d64 = 0 mm, d653_d74_d65 = 0 mm, d654_d75 = 0 mm, d655_d76 = 9.5 mm, d656_d77 = 0 mm, d657_d78 = 0 mm, d658_d79 = 0 mm, d659_d81 = 0 mm, d660_d82 = 0 mm, d661_d83_d6 = 0 mm, d662_d84_d7 = -12.858 mm, d663_d85_d8 = -15 mm, d664_d86_d0 = 0 mm, d665_d87_d1 = 0 deg, d666_d88_d3 = 0 mm, d667_d89_d4 = 5 mm, d668_d90_d5 = 0 deg, d669_d5 = 0 deg, d670_d6 = 0 mm, d671_d7 = 0 mm, d672_d8 = 0 deg, d673_d9 = 0 mm, d674_d10 = 0 mm, d675_d11 = 0 deg, d676_d29_d6 = 0 mm, d677_d30_d7 = 0 mm, d678_d31_d8 = 0 deg, d679_d32_d9 = 0 mm, d680_d33_d10 = 0 mm, d681_d34_d11 = 0 deg, d682_d37 = 0 mm, d683_d40_d3 = 0 mm, d684_d41_d4 = 0 deg, d685_d42_d5 = 0 deg, d686_d43_d0 = 0 mm, d687_d44_d1 = 0 mm, d688_d45_d2 = 0 mm, d689_d48 = 0 mm, d690_d0 = 0 mm, d691_d1 = 0 mm, d692_d2 = 0 mm, d693_d3 = 0 mm, d694_d4 = 0 deg, d102_d31 = 0 mm, d103_d32 = 7 mm, d104_d33 = 0 mm, d105_d34 = 0 mm, d705_d35 = 0 mm, d706_d36 = 31 mm, d707_d37 = 0 mm, d109_d23 = 0 mm, d110_d24 = 0 mm, d111_d25 = 0 mm, d112_d26 = 0 mm, d113_d27 = 7 mm, d114_d28 = 0 mm, d115_d30 = 0 mm, d715_d116 = 0 mm, d716_d117 = 0 mm, d717_d118 = 0 mm, d718_d119 = 0 mm, susp_angle = 108 deg
